# Autodesk Inventor assembly: ForeArm_diagonal
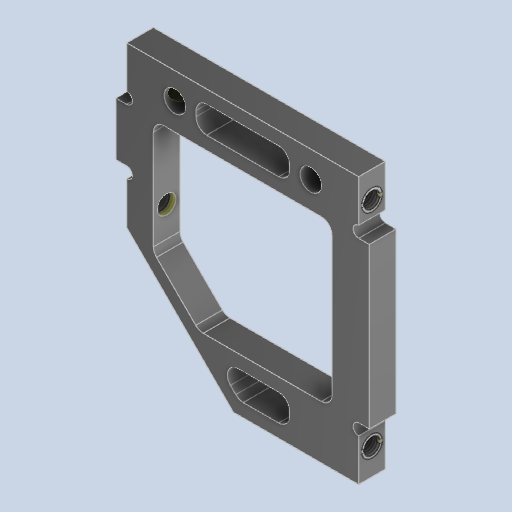
[picture p0: Inventor's stored thumbnail of the model, 512x512]
Saved by Autodesk Inventor 2022.5 (Build 265521000, 521)
## iProperties
Created: 2023-06-02
Part Number: ForeArm_diagonal
Document SubType Name: Assembly
Designer: Masato Kubotera
Author: Masato Kubotera
## Documents named in this file (3)
- C:\Users\Masato\Documents\Inventor\SUSTAINA-OP\ModelingFiles\UpperBody\Arm\ForeArm_diagonal.iam
- C:\Users\Masato\Documents\Inventor\SUSTAINA-OP\ModelingFiles\UpperBody\Arm\ForeArm_diagonal.ipt
- C:\Users\Masato\Documents\Inventor\SUSTAINA-OP\ModelingFiles\COTS\InsertNut\IRU-304S.ipt
## Components (5 placed, 2 different names)
1. ForeArm_diagonal:1 — Flush:1, Flush:2, Flush:3, Insert:1, Insert:2, Insert:3, Insert:4
2. IRU-304S:1 — Insert:1
3. IRU-304S:2 — Insert:2
4. IRU-304S:3 — Insert:3
5. IRU-304S:4 — Insert:4
## Relationships (7: Insert 4, Flush 3)
- Flush:1: ForeArm_diagonal:1
- Flush:2: ForeArm_diagonal:1
- Flush:3: ForeArm_diagonal:1
- Insert:1: ForeArm_diagonal:1 ↔ IRU-304S:1
- Insert:2: ForeArm_diagonal:1 ↔ IRU-304S:2
- Insert:3: ForeArm_diagonal:1 ↔ IRU-304S:3
- Insert:4: ForeArm_diagonal:1 ↔ IRU-304S:4
